# Autodesk Inventor assembly: Base
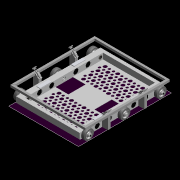
[picture p0: Inventor's stored thumbnail of the model, 180x180]
Saved by Autodesk Inventor 2014 SP1 (Build 180222100, 222)
## iProperties
Created: 2013-11-29
Part Number: Base
Document SubType Name: Assembly
Designer: Rauhul Varma
Author: Rauhul Varma
## Documents named in this file (23)
- C:\Users\Rauhul Varma\Desktop\2014 Base\Base.iam
- C:\Users\Rauhul Varma\Desktop\2014 Base\Tube.ipt
- C:\Users\Rauhul Varma\Desktop\2014 Base\Live Axle Assembly.iam
- C:\Users\Rauhul Varma\Desktop\2014 Base\Plastic Plug.ipt
- C:\Users\Rauhul Varma\Desktop\2014 Base\FR8-2RS Bearing.ipt
- C:\Users\Rauhul Varma\Desktop\2014 Base\3.5 in by 1.25 in Colson Wheel.ipt
- C:\Users\Rauhul Varma\Desktop\2014 Base\Colson Hub.ipt
- C:\Users\Rauhul Varma\Desktop\2014 Base\Center Axle.ipt
- C:\Users\Rauhul Varma\Desktop\2014 Base\22T 5mm GT2 Pulley.ipt
- C:\Users\Rauhul Varma\Desktop\2014 Base\Belly Pan.ipt
- C:\Users\Rauhul Varma\Desktop\2014 Base\150T 5mm GT2 Belt.ipt
- C:\Users\Rauhul Varma\Desktop\2014 Base\Bumper Rail Stand Bottom Cap.ipt
- C:\Users\Rauhul Varma\Desktop\2014 Base\Bumper Rail Stand.ipt
- C:\Users\Rauhul Varma\Desktop\2014 Base\Bumper Rail Stand Top Cap.ipt
- C:\Users\Rauhul Varma\Desktop\2014 Base\Bumper Rail Side.ipt
- C:\Users\Rauhul Varma\Desktop\2014 Base\Bumper Rail Cross.ipt
- C:\Users\Rauhul Varma\Desktop\2014 Base\Belt Aligners.ipt
- C:\Users\Rauhul Varma\Desktop\2014 Base\Tube Reversed.ipt
- C:\Users\Rauhul Varma\Desktop\2014 Base\Bolt On Cross Support.ipt
- C:\Users\Rauhul Varma\Desktop\2014 Base\Latch.iam
- C:\Users\Rauhul Varma\Desktop\2014 Base\Bumpers.iam
- C:\Users\Rauhul Varma\Desktop\2014 Base\Belt Aligner MagLock.ipt
- C:\Users\Rauhul Varma\Desktop\2014 Base\MagLock Magnet.ipt
## Components (70 placed, 22 different names)
1. Latch:1 [sub-assembly] — Mate:184, Mate:185, Mate:186, Mate:189, Mate:191, Mate:192
2. Latch:2 [sub-assembly] — Mate:193, Mate:194, Mate:195, Mate:196
3. Latch:3 [sub-assembly] — Mate:199, Mate:200, Mate:201, Mate:202, Mate:203
4. Latch:4 [sub-assembly] — Mate:204, Mate:205, Mate:206, Mate:207
5. Bumpers:1 [sub-assembly] — Mate:187, Mate:188, Flush:34, Mate:189, Mate:191, Mate:192, Mate:193, Mate:195, Mate:202, Mate:203, Mate:206, Mate:207
6. Belt Aligner MagLock:1 — Flush:38, Mate:230, Mate:231
7. Belt Aligner MagLock:2 — Flush:37, Flush:38, Mate:232, Mate:235
8. Belt Aligner MagLock:3 — Flush:36, Flush:37, Mate:233, Mate:234
9. Belt Aligner MagLock:4 — Flush:36, Mate:219, Mate:220, Mate:221, Mate:222, Mate:223, Mate:224, Mate:227, Mate:228, Mate:229
10. MagLock Magnet:1 — Mate:223, Mate:224, Mate:229
11. MagLock Magnet:2 — Mate:222, Mate:227, Mate:228
12. Bolt On Cross Support:2 — Mate:210, Mate:211, Mate:212
13. Tube:1 — Mate:11, Mate:12, Mate:13, Mate:14, Mate:35, Mate:36, Mate:37, Mate:38, Mate:39, Mate:40, Mate:41, Mate:42, Mate:43, Mate:44, Mate:45, Mate:46, Mate:47, Mate:48, Mate:85, Mate:86, Mate:94, Mate:95, Mate:121, Mate:122, Mate:136, Mate:151, Mate:152, Mate:159, Mate:160, Mate:161, Mate:162, Mate:208, Mate:218, Mate:232, Mate:233, Mate:234, Mate:235
14. Tube Reversed:1 — Mate:141, Mate:145, Mate:146, Mate:147, Mate:148, Mate:149, Mate:150, Mate:153, Mate:154, Mate:156, Mate:157, Mate:165, Mate:166, Mate:167, Mate:168, Mate:169, Mate:170, Mate:171, Mate:172, Mate:173, Mate:174, Mate:175, Mate:176, Mate:177, Mate:178, Mate:179, Mate:180, Flush:35, Mate:211, Mate:214, Mate:217, Mate:219, Mate:220, Mate:221, Mate:230, Mate:231
15. Bolt On Cross Support:1 — Mate:215, Mate:216, Mate:217, Mate:218
16. Belly Pan:1 — Mate:136, Flush:25, Flush:26, Flush:27, Flush:28, Mate:141, Flush:33, Mate:208, Flush:35, Mate:210, Mate:212, Mate:214, Mate:215, Mate:216
17. Plastic Plug:1 — Mate:173, Mate:177
18. Plastic Plug:2 — Mate:166, Mate:171
19. Plastic Plug:3 — Mate:167, Mate:170
20. Plastic Plug:4 — Mate:165, Mate:172
21. Plastic Plug:5 — Mate:168, Mate:169
22. Plastic Plug:6 — Mate:174, Mate:178
23. Plastic Plug:7 — Mate:175, Mate:179
24. Plastic Plug:8 — Mate:176, Mate:180
25. Plastic Plug:9 — Mate:40, Mate:44
26. Plastic Plug:10 — Mate:39, Mate:43
27. Plastic Plug:11 — Mate:42, Mate:46
28. Plastic Plug:12 — Mate:41, Mate:45
29. Plastic Plug:13 — Mate:38, Mate:162
30. Plastic Plug:14 — Mate:37, Mate:161
31. Plastic Plug:15 — Mate:36, Mate:160
32. Plastic Plug:16 — Mate:35, Mate:159
33. 150T 5mm GT2 Belt:1 — Mate:75, Mate:76, Flush:2
34. 150T 5mm GT2 Belt:2 — Mate:73, Mate:74, Flush:3
35. 150T 5mm GT2 Belt:3 — Mate:78, Mate:79, Flush:5
36. 150T 5mm GT2 Belt:4 — Mate:77, Mate:80, Flush:4
37. Live Axle Assembly:1 [sub-assembly] — Mate:74, Mate:147, Mate:148
38. Live Axle Assembly:2 [sub-assembly] — Mate:76, Mate:149, Mate:150
39. Live Axle Assembly:3 [sub-assembly] — Mate:11, Mate:12, Mate:79
40. Live Axle Assembly:4 [sub-assembly] — Mate:13, Mate:14, Mate:80
41. FR8-2RS Bearing:1 — Mate:47, Mate:48, Mate:55, Mate:56, Mate:62, Mate:64, Mate:66, Mate:70, Mate:77, Mate:78
42. FR8-2RS Bearing:2 — Mate:57, Mate:58, Mate:59, Mate:60, Mate:65, Mate:68, Mate:73, Mate:75, Mate:146
43. 3.5 in by 1.25 in Colson Wheel:1 — Mate:53, Mate:54
44. Colson Hub:1 — Mate:53, Mate:54, Mate:57, Mate:58, Mate:61
45. 3.5 in by 1.25 in Colson Wheel:2 — Mate:51, Mate:52
46. Colson Hub:2 — Mate:51, Mate:52, Mate:55, Mate:56, Mate:63
47. Center Axle:1 — Mate:62, Mate:63, Mate:64, Mate:69
48. Center Axle:2 — Mate:59, Mate:60, Mate:61, Mate:67
49. 22T 5mm GT2 Pulley:1 — Mate:66, Mate:69, Mate:70, Flush:4, Flush:5
50. 22T 5mm GT2 Pulley:2 — Mate:65, Mate:67, Mate:68, Flush:2, Flush:3, Mate:145
51. Bumper Rail Stand:1 — Mate:85, Mate:86, Mate:87, Flush:7, Mate:88, Mate:96, Mate:97, Mate:137, Flush:23, Flush:24, Flush:30, Mate:164
52. Bumper Rail Stand Top Cap:1 — Mate:87, Flush:7, Mate:88, Mate:184, Mate:185, Mate:186
53. Bumper Rail Stand:2 — Mate:94, Mate:95, Mate:133, Mate:138, Flush:21, Flush:22, Flush:29, Mate:163
54. Bumper Rail Stand Top Cap:2 — Mate:194, Mate:196
55. Bumper Rail Side:1 — Mate:96, Mate:97, Mate:116, Flush:13, Mate:117, Mate:120, Flush:15, Mate:133
56. Bumper Rail Stand:3 — Mate:140, Flush:17, Flush:18, Flush:30, Mate:155
57. Bumper Rail Stand Top Cap:3 — Mate:204, Mate:205
58. Bumper Rail Stand:4 — Mate:110, Mate:111, Mate:139, Flush:19, Flush:20, Flush:29, Mate:158
59. Bumper Rail Stand Top Cap:4 — Mate:199, Mate:200, Mate:201
60. Bumper Rail Side:2 — Mate:110, Mate:111, Mate:115, Mate:118, Flush:14, Mate:119, Mate:188
61. Bumper Rail Cross:1 — Mate:119, Mate:120, Flush:15, Mate:187
62. Bumper Rail Cross:2 — Mate:115, Mate:116, Flush:13, Mate:117, Mate:118, Flush:14
63. Bumper Rail Stand Bottom Cap:1 — Mate:137, Flush:23, Flush:24, Flush:25
64. Bumper Rail Stand Bottom Cap:2 — Mate:138, Flush:21, Flush:22, Flush:26
65. Bumper Rail Stand Bottom Cap:3 — Mate:140, Flush:17, Flush:18, Flush:28
66. Bumper Rail Stand Bottom Cap:4 — Mate:139, Flush:19, Flush:20, Flush:27
67. Belt Aligners:1 — Mate:121, Mate:151, Mate:164
68. Belt Aligners:2 — Mate:122, Mate:152, Mate:163
69. Belt Aligners:3 — Mate:156, Mate:157, Mate:158
70. Belt Aligners:4 — Mate:153, Mate:154, Mate:155
## Relationships (191: Mate 160, Flush 31)
- Mate:11: Tube:1 ↔ Live Axle Assembly:3
- Mate:12: Tube:1 ↔ Live Axle Assembly:3
- Mate:13: Tube:1 ↔ Live Axle Assembly:4
- Mate:14: Tube:1 ↔ Live Axle Assembly:4
- Mate:35: Tube:1 ↔ Plastic Plug:16
- Mate:36: Tube:1 ↔ Plastic Plug:15
- Mate:37: Tube:1 ↔ Plastic Plug:14
- Mate:38: Tube:1 ↔ Plastic Plug:13
- Mate:39: Tube:1 ↔ Plastic Plug:10
- Mate:40: Tube:1 ↔ Plastic Plug:9
- Mate:41: Tube:1 ↔ Plastic Plug:12
- Mate:42: Tube:1 ↔ Plastic Plug:11
- Mate:43: Tube:1 ↔ Plastic Plug:10
- Mate:44: Tube:1 ↔ Plastic Plug:9
- Mate:45: Tube:1 ↔ Plastic Plug:12
- Mate:46: Tube:1 ↔ Plastic Plug:11
- Mate:47: Tube:1 ↔ FR8-2RS Bearing:1
- Mate:48: Tube:1 ↔ FR8-2RS Bearing:1
- Mate:51: 3.5 in by 1.25 in Colson Wheel:2 ↔ Colson Hub:2
- Mate:52: 3.5 in by 1.25 in Colson Wheel:2 ↔ Colson Hub:2
- Mate:53: 3.5 in by 1.25 in Colson Wheel:1 ↔ Colson Hub:1
- Mate:54: 3.5 in by 1.25 in Colson Wheel:1 ↔ Colson Hub:1
- Mate:55: FR8-2RS Bearing:1 ↔ Colson Hub:2
- Mate:56: FR8-2RS Bearing:1 ↔ Colson Hub:2
- Mate:57: FR8-2RS Bearing:2 ↔ Colson Hub:1
- Mate:58: FR8-2RS Bearing:2 ↔ Colson Hub:1
- Mate:59: FR8-2RS Bearing:2 ↔ Center Axle:2
- Mate:60: FR8-2RS Bearing:2 ↔ Center Axle:2
- Mate:61: Colson Hub:1 ↔ Center Axle:2
- Mate:62: FR8-2RS Bearing:1 ↔ Center Axle:1
- Mate:63: Colson Hub:2 ↔ Center Axle:1
- Mate:64: FR8-2RS Bearing:1 ↔ Center Axle:1
- Mate:65: FR8-2RS Bearing:2 ↔ 22T 5mm GT2 Pulley:2
- Mate:66: FR8-2RS Bearing:1 ↔ 22T 5mm GT2 Pulley:1
- Mate:67: Center Axle:2 ↔ 22T 5mm GT2 Pulley:2
- Mate:68: FR8-2RS Bearing:2 ↔ 22T 5mm GT2 Pulley:2
- Mate:69: Center Axle:1 ↔ 22T 5mm GT2 Pulley:1
- Mate:70: FR8-2RS Bearing:1 ↔ 22T 5mm GT2 Pulley:1
- Mate:73: 150T 5mm GT2 Belt:2 ↔ FR8-2RS Bearing:2
- Mate:74: 150T 5mm GT2 Belt:2 ↔ Live Axle Assembly:1
- Mate:75: 150T 5mm GT2 Belt:1 ↔ FR8-2RS Bearing:2
- Mate:76: 150T 5mm GT2 Belt:1 ↔ Live Axle Assembly:2
- Flush:2 (-2.4354 mm): 150T 5mm GT2 Belt:1 ↔ 22T 5mm GT2 Pulley:2
- Flush:3 (2.4354 mm): 150T 5mm GT2 Belt:2 ↔ 22T 5mm GT2 Pulley:2
- Mate:77: 150T 5mm GT2 Belt:4 ↔ FR8-2RS Bearing:1
- Mate:78: 150T 5mm GT2 Belt:3 ↔ FR8-2RS Bearing:1
- Mate:79: 150T 5mm GT2 Belt:3 ↔ Live Axle Assembly:3
- Mate:80: 150T 5mm GT2 Belt:4 ↔ Live Axle Assembly:4
- Flush:4 (2.4354 mm): 150T 5mm GT2 Belt:4 ↔ 22T 5mm GT2 Pulley:1
- Flush:5 (2.4354 mm): 150T 5mm GT2 Belt:3 ↔ 22T 5mm GT2 Pulley:1
- Mate:85: Tube:1 ↔ Bumper Rail Stand:1
- Mate:86 (25.4 mm): Tube:1 ↔ Bumper Rail Stand:1
- Mate:87: Bumper Rail Stand:1 ↔ Bumper Rail Stand Top Cap:1
- Flush:7: Bumper Rail Stand:1 ↔ Bumper Rail Stand Top Cap:1
- Mate:88: Bumper Rail Stand:1 ↔ Bumper Rail Stand Top Cap:1
- [Mate]: Bumper Rail Stand:2 ↔ Bumper Rail Stand Top Cap:2
- [Flush]: Bumper Rail Stand:2 ↔ Bumper Rail Stand Top Cap:2
- [Mate]: Bumper Rail Stand:2 ↔ Bumper Rail Stand Top Cap:2
- Mate:94: Tube:1 ↔ Bumper Rail Stand:2
- Mate:95 (25.4 mm): Tube:1 ↔ Bumper Rail Stand:2
- Mate:96: Bumper Rail Stand:1 ↔ Bumper Rail Side:1
- Mate:97: Bumper Rail Stand:1 ↔ Bumper Rail Side:1
- [Mate]: Bumper Rail Stand:3 ↔ Bumper Rail Stand Top Cap:3
- [Flush]: Bumper Rail Stand:3 ↔ Bumper Rail Stand Top Cap:3
- [Mate]: Bumper Rail Stand:3 ↔ Bumper Rail Stand Top Cap:3
- [Mate]: Bumper Rail Stand:4 ↔ Bumper Rail Stand Top Cap:4
- [Flush]: Bumper Rail Stand:4 ↔ Bumper Rail Stand Top Cap:4
- [Mate]: Bumper Rail Stand:4 ↔ Bumper Rail Stand Top Cap:4
- [Mate]: Bumper Rail Stand:3 ↔ Bumper Rail Side:2
- [Mate]: Bumper Rail Stand:3 ↔ Bumper Rail Side:2
- Mate:110: Bumper Rail Stand:4 ↔ Bumper Rail Side:2
- Mate:111: Bumper Rail Stand:4 ↔ Bumper Rail Side:2
- Mate:115: Bumper Rail Side:2 ↔ Bumper Rail Cross:2
- Mate:116: Bumper Rail Side:1 ↔ Bumper Rail Cross:2
- Flush:13: Bumper Rail Side:1 ↔ Bumper Rail Cross:2
- Mate:117: Bumper Rail Side:1 ↔ Bumper Rail Cross:2
- Mate:118: Bumper Rail Side:2 ↔ Bumper Rail Cross:2
- Flush:14: Bumper Rail Side:2 ↔ Bumper Rail Cross:2
- Mate:119: Bumper Rail Side:2 ↔ Bumper Rail Cross:1
- Mate:120: Bumper Rail Side:1 ↔ Bumper Rail Cross:1
- Flush:15: Bumper Rail Side:1 ↔ Bumper Rail Cross:1
- Mate:121: Tube:1 ↔ Belt Aligners:1
- Mate:122: Tube:1 ↔ Belt Aligners:2
- Mate:133: Bumper Rail Stand:2 ↔ Bumper Rail Side:1
- Mate:136: Tube:1 ↔ Belly Pan:1
- Mate:137: Bumper Rail Stand:1 ↔ Bumper Rail Stand Bottom Cap:1
- Mate:138: Bumper Rail Stand:2 ↔ Bumper Rail Stand Bottom Cap:2
- Mate:139: Bumper Rail Stand:4 ↔ Bumper Rail Stand Bottom Cap:4
- Mate:140: Bumper Rail Stand:3 ↔ Bumper Rail Stand Bottom Cap:3
- Flush:17: Bumper Rail Stand:3 ↔ Bumper Rail Stand Bottom Cap:3
- Flush:18: Bumper Rail Stand:3 ↔ Bumper Rail Stand Bottom Cap:3
- Flush:19: Bumper Rail Stand:4 ↔ Bumper Rail Stand Bottom Cap:4
- Flush:20: Bumper Rail Stand:4 ↔ Bumper Rail Stand Bottom Cap:4
- Flush:21: Bumper Rail Stand:2 ↔ Bumper Rail Stand Bottom Cap:2
- Flush:22: Bumper Rail Stand:2 ↔ Bumper Rail Stand Bottom Cap:2
- Flush:23: Bumper Rail Stand:1 ↔ Bumper Rail Stand Bottom Cap:1
- Flush:24: Bumper Rail Stand:1 ↔ Bumper Rail Stand Bottom Cap:1
- Flush:25: Belly Pan:1 ↔ Bumper Rail Stand Bottom Cap:1
- Flush:26: Belly Pan:1 ↔ Bumper Rail Stand Bottom Cap:2
- Flush:27: Belly Pan:1 ↔ Bumper Rail Stand Bottom Cap:4
- Flush:28: Belly Pan:1 ↔ Bumper Rail Stand Bottom Cap:3
- Mate:141: Tube Reversed:1 ↔ Belly Pan:1
- Mate:145: Tube Reversed:1 ↔ 22T 5mm GT2 Pulley:2
- Mate:146: Tube Reversed:1 ↔ FR8-2RS Bearing:2
- Mate:147: Tube Reversed:1 ↔ Live Axle Assembly:1
- Mate:148: Tube Reversed:1 ↔ Live Axle Assembly:1
- Mate:149: Tube Reversed:1 ↔ Live Axle Assembly:2
- Mate:150: Tube Reversed:1 ↔ Live Axle Assembly:2
- Flush:29: Bumper Rail Stand:2 ↔ Bumper Rail Stand:4
- Flush:30: Bumper Rail Stand:1 ↔ Bumper Rail Stand:3
- Mate:151: Tube:1 ↔ Belt Aligners:1
- Mate:152: Tube:1 ↔ Belt Aligners:2
- Mate:153: Tube Reversed:1 ↔ Belt Aligners:4
- Mate:154: Tube Reversed:1 ↔ Belt Aligners:4
- Mate:155: Bumper Rail Stand:3 ↔ Belt Aligners:4
- Mate:156: Tube Reversed:1 ↔ Belt Aligners:3
- Mate:157: Tube Reversed:1 ↔ Belt Aligners:3
- Mate:158: Bumper Rail Stand:4 ↔ Belt Aligners:3
- Mate:159: Tube:1 ↔ Plastic Plug:16
- Mate:160: Tube:1 ↔ Plastic Plug:15
- Mate:161: Tube:1 ↔ Plastic Plug:14
- Mate:162: Tube:1 ↔ Plastic Plug:13
- Mate:163: Bumper Rail Stand:2 ↔ Belt Aligners:2
- Mate:164: Bumper Rail Stand:1 ↔ Belt Aligners:1
- Mate:165: Tube Reversed:1 ↔ Plastic Plug:4
- Mate:166: Tube Reversed:1 ↔ Plastic Plug:2
- Mate:167: Tube Reversed:1 ↔ Plastic Plug:3
- Mate:168: Tube Reversed:1 ↔ Plastic Plug:5
- Mate:169: Tube Reversed:1 ↔ Plastic Plug:5
- Mate:170: Tube Reversed:1 ↔ Plastic Plug:3
- Mate:171: Tube Reversed:1 ↔ Plastic Plug:2
- Mate:172: Tube Reversed:1 ↔ Plastic Plug:4
- Mate:173: Tube Reversed:1 ↔ Plastic Plug:1
- Mate:174: Tube Reversed:1 ↔ Plastic Plug:6
- Mate:175: Tube Reversed:1 ↔ Plastic Plug:7
- Mate:176: Tube Reversed:1 ↔ Plastic Plug:8
- Mate:177: Tube Reversed:1 ↔ Plastic Plug:1
- Mate:178: Tube Reversed:1 ↔ Plastic Plug:6
- Mate:179: Tube Reversed:1 ↔ Plastic Plug:7
- Mate:180: Tube Reversed:1 ↔ Plastic Plug:8
- Mate:184: Latch:1 ↔ Bumper Rail Stand Top Cap:1
- Mate:185: Latch:1 ↔ Bumper Rail Stand Top Cap:1
- Mate:186: Latch:1 ↔ Bumper Rail Stand Top Cap:1
- Mate:187: Bumpers:1 ↔ Bumper Rail Cross:1
- Mate:188: Bumpers:1 ↔ Bumper Rail Side:2
- Flush:33 (17.5133 mm): Belly Pan:1
- Flush:34 (50.8 mm): Bumpers:1
- Mate:189: Latch:1 ↔ Bumpers:1
- Mate:191: Latch:1 ↔ Bumpers:1
- Mate:192: Latch:1 ↔ Bumpers:1
- Mate:193: Latch:2 ↔ Bumpers:1
- Mate:194: Latch:2 ↔ Bumper Rail Stand Top Cap:2
- Mate:195: Latch:2 ↔ Bumpers:1
- Mate:196: Latch:2 ↔ Bumper Rail Stand Top Cap:2
- Mate:199: Latch:3 ↔ Bumper Rail Stand Top Cap:4
- Mate:200: Latch:3 ↔ Bumper Rail Stand Top Cap:4
- Mate:201: Latch:3 ↔ Bumper Rail Stand Top Cap:4
- Mate:202: Latch:3 ↔ Bumpers:1
- Mate:203: Latch:3 ↔ Bumpers:1
- Mate:204: Latch:4 ↔ Bumper Rail Stand Top Cap:3
- Mate:205: Latch:4 ↔ Bumper Rail Stand Top Cap:3
- Mate:206: Latch:4 ↔ Bumpers:1
- Mate:207: Latch:4 ↔ Bumpers:1
- Mate:208: Tube:1 ↔ Belly Pan:1
- Flush:35: Tube Reversed:1 ↔ Belly Pan:1
- Mate:210: Bolt On Cross Support:2 ↔ Belly Pan:1
- Mate:211: Bolt On Cross Support:2 ↔ Tube Reversed:1
- Mate:212: Bolt On Cross Support:2 ↔ Belly Pan:1
- Mate:214: Tube Reversed:1 ↔ Belly Pan:1
- Mate:215: Bolt On Cross Support:1 ↔ Belly Pan:1
- Mate:216: Bolt On Cross Support:1 ↔ Belly Pan:1
- Mate:217: Tube Reversed:1 ↔ Bolt On Cross Support:1
- Mate:218: Tube:1 ↔ Bolt On Cross Support:1
- Flush:36: Belt Aligner MagLock:3 ↔ Belt Aligner MagLock:4
- Flush:37: Belt Aligner MagLock:2 ↔ Belt Aligner MagLock:3
- Flush:38: Belt Aligner MagLock:1 ↔ Belt Aligner MagLock:2
- Mate:219: Belt Aligner MagLock:4 ↔ Tube Reversed:1
- Mate:220: Belt Aligner MagLock:4 ↔ Tube Reversed:1
- Mate:221 (-11.1125 mm): Belt Aligner MagLock:4 ↔ Tube Reversed:1
- Mate:222: Belt Aligner MagLock:4 ↔ MagLock Magnet:2
- Mate:223: Belt Aligner MagLock:4 ↔ MagLock Magnet:1
- Mate:224: Belt Aligner MagLock:4 ↔ MagLock Magnet:1
- Mate:227: Belt Aligner MagLock:4 ↔ MagLock Magnet:2
- Mate:228: Belt Aligner MagLock:4 ↔ MagLock Magnet:2
- Mate:229: Belt Aligner MagLock:4 ↔ MagLock Magnet:1
- Mate:230: Belt Aligner MagLock:1 ↔ Tube Reversed:1
- Mate:231 (3.175 mm): Belt Aligner MagLock:1 ↔ Tube Reversed:1
- Mate:232: Belt Aligner MagLock:2 ↔ Tube:1
- Mate:233: Belt Aligner MagLock:3 ↔ Tube:1
- Mate:234 (3.175 mm): Belt Aligner MagLock:3 ↔ Tube:1
- Mate:235 (3.175 mm): Belt Aligner MagLock:2 ↔ Tube:1
## Named parameters: d98_d92 = 0 mm, d99_d93 = 0 mm, d100_d94 = 0 mm, d110_d92 = 0 mm, d111_d93 = 0 mm, d112_d94 = 0 mm, d116_d98_d92 = 0 mm, d117_d99_d93 = 0 mm, d118_d100_d94 = 0 mm, d119_d104 = 0 mm, d120_d105 = 0 mm
